# Autodesk Inventor assembly: LCD_with_bracket
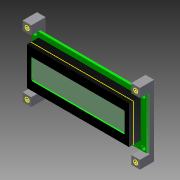
[picture p0: Inventor's stored thumbnail of the model, 180x180]
Saved by Autodesk Inventor 2015 (Build 190159000, 159)
## iProperties
Created: 2015-03-09
Part Number: LCD_with_bracket
Document SubType Name: Assembly
Designer: ChristopherEvan
Author: ChristopherEvan
## Documents named in this file (3)
- C:\Users\ChristopherEvan\Documents\Inventor\MAKE\Enclosure\LCD\LCD_with_bracket.iam
- C:\Users\ChristopherEvan\Documents\Inventor\MAKE\Enclosure\LCD\LCD.ipt
- C:\Users\ChristopherEvan\Documents\Inventor\MAKE\Enclosure\LCD\LCD_bracket.ipt
## Components (2 placed, 2 different names)
1. LCD:1 — Mate:1, Mate:2, Mate:3, Mate:4
2. LCD_bracket:1 — Mate:1, Mate:2, Mate:3, Mate:4
## Relationships (4: Mate 4)
- Mate:1: LCD:1 ↔ LCD_bracket:1
- Mate:2: LCD:1 ↔ LCD_bracket:1
- Mate:3: LCD:1 ↔ LCD_bracket:1
- Mate:4: LCD:1 ↔ LCD_bracket:1
